# Autodesk Inventor assembly: Large2020Gantry
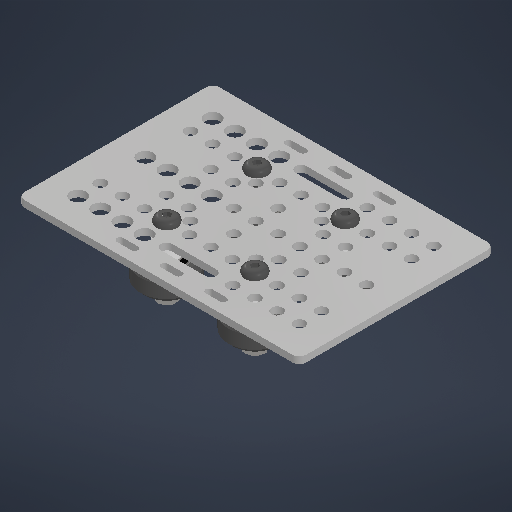
[picture p0: Inventor's stored thumbnail of the model, 512x512]
Saved by Autodesk Inventor 2027.1 (Build 311270010, 270A)
## iProperties
Created: 2026-10-03
Part Number: Large2020Gantry
Document SubType Name: Assembly
Designer: SDS Scholar
Author: SDS Scholar
## Documents named in this file (3)
- E:\Apps\AutodeskInventor\University\MCT333_Design1\OnTheShelf\VSoltGantrySetAllSizes\Large2020Gantry.iam
- E:\Apps\AutodeskInventor\University\MCT333_Design1\OnTheShelf\VSoltGantrySetAllSizes\v-slot-gantry-plate-20-80mm\V-Slot Gantry Plate 20-80mm\V-Slot Gantry Plate 20-80mm.ipt
- E:\Apps\AutodeskInventor\University\MCT333_Design1\OnTheShelf\VSoltGantrySetAllSizes\solid-v-wheel-kit-b-size\SVWB.iam
## Components (5 placed, 2 different names)
1. V-Slot Gantry Plate 20-80mm:1 — Mate:1, Mate:2, Mate:3, Mate:4, Mate:5, Mate:6, Mate:7, Mate:8, Mate:9, Mate:10, Mate:11
2. SVWB:1 [sub-assembly] — Mate:6, Mate:8
3. SVWB:2 [sub-assembly] — Mate:5, Mate:10
4. SVWB:3 [sub-assembly] — Mate:4, Mate:11
5. SVWB:4 [sub-assembly] — Mate:7, Mate:9
## Relationships (11: Mate 11)
- Mate:1: V-Slot Gantry Plate 20-80mm:1
- Mate:2: V-Slot Gantry Plate 20-80mm:1
- Mate:3: V-Slot Gantry Plate 20-80mm:1
- Mate:4: V-Slot Gantry Plate 20-80mm:1 ↔ SVWB:3
- Mate:5: V-Slot Gantry Plate 20-80mm:1 ↔ SVWB:2
- Mate:6: V-Slot Gantry Plate 20-80mm:1 ↔ SVWB:1
- Mate:7: V-Slot Gantry Plate 20-80mm:1 ↔ SVWB:4
- Mate:8: V-Slot Gantry Plate 20-80mm:1 ↔ SVWB:1
- Mate:9: V-Slot Gantry Plate 20-80mm:1 ↔ SVWB:4
- Mate:10: V-Slot Gantry Plate 20-80mm:1 ↔ SVWB:2
- Mate:11: V-Slot Gantry Plate 20-80mm:1 ↔ SVWB:3
